# Autodesk Inventor assembly: Dual Redline_2_1-2inHex
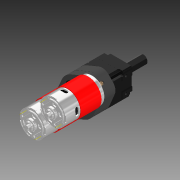
[picture p0: Inventor's stored thumbnail of the model, 180x180]
Saved by Autodesk Inventor 2021 (Build 250183000, 183)
## iProperties
Created: 2018-08-19
Part Number: Dual Redline_2_1-2inHex
Document SubType Name: Assembly
Mass: 1123.04 g
Surface Area: 1203.25 cm^2
Volume: 285.054 cm^3
Density: 3.93975 g/cm^3
## Documents named in this file (10)
- D:\FIRST\Design\CollabPartsLib\Motors\FRC\Versaplanetary\VersaPlanetary\Dual Redline, 2 Stages, 1-2in Hex Output.iam
- D:\FIRST\Design\CollabPartsLib\Motors\FRC\Versaplanetary\V2 Stages\V2 Output Stage.iam
- D:\FIRST\Design\CollabPartsLib\Motors\FRC\Versaplanetary\Intermediate Stages\Ring Gear.ipt
- D:\FIRST\Design\CollabPartsLib\Motors\FRC\Versaplanetary\V2 Stages\Dual Input Stage.iam
- D:\FIRST\Design\CollabPartsLib\Motors\FRC\Versaplanetary\Screws\8-32 x 1.75in Screw.ipt
- D:\FIRST\Design\CollabPartsLib\Power Transfer\Bearings\6902ZZ.ipt
- D:\FIRST\Design\CollabPartsLib\Motors\FRC\Versaplanetary\V2 Stages\V2 Output Stage\VP V2 Output Stage 1-2in Hex.iam
- D:\FIRST\Design\CollabPartsLib\Power Transfer\Bearings.ipt
- D:\FIRST\Design\CollabPartsLib\Motors\FRC\Versaplanetary\VersaPlanetary.iam
- D:\FIRST\Design\CollabPartsLib\Motors\FRC\Versaplanetary\V2 Stages\Dual Input Stage\VP Dual Redline Input.iam
## Components (8 placed, 6 different names)
1. VP V2 Output Stage 1-2in Hex:1 [sub-assembly] — Insert:1, Flush:3, Flush:6, 2StageDualInputMate1, 2StageDualInputMate3, Insert:25
2. Ring Gear 1 — Insert:1, Insert:2, Flush:1, Flush:3
3. Ring Gear 2 — Insert:2, Flush:1, Flush:6, 2StageDualInputMate2
4. VP Dual Redline Input:1 [sub-assembly] — 2StageDualInputMate1, 2StageDualInputMate2, 2StageDualInputMate3, Insert:20, Insert:21
5. 8-32 x 1.75in Screw:5 — Insert:21
6. 8-32 x 1.75in Screw:6 — Insert:20
7. 6902ZZ:1
8. 6902ZZ:2 — Insert:25
## Relationships (11: Insert 5, Flush 3, Mate 3)
- Insert:1: VP V2 Output Stage 1-2in Hex:1 ↔ Ring Gear 1
- Insert:2: Ring Gear 1 ↔ Ring Gear 2
- Flush:1: Ring Gear 1 ↔ Ring Gear 2
- Flush:3: VP V2 Output Stage 1-2in Hex:1 ↔ Ring Gear 1
- Flush:6: VP V2 Output Stage 1-2in Hex:1 ↔ Ring Gear 2
- 2StageDualInputMate1 [Mate]: VP V2 Output Stage 1-2in Hex:1 ↔ VP Dual Redline Input:1
- 2StageDualInputMate2 [Mate]: Ring Gear 2 ↔ VP Dual Redline Input:1
- 2StageDualInputMate3 [Mate]: VP V2 Output Stage 1-2in Hex:1 ↔ VP Dual Redline Input:1
- Insert:20: VP Dual Redline Input:1 ↔ 8-32 x 1.75in Screw:6
- Insert:21: VP Dual Redline Input:1 ↔ 8-32 x 1.75in Screw:5
- Insert:25: VP V2 Output Stage 1-2in Hex:1 ↔ 6902ZZ:2
